# Autodesk Inventor assembly: Assembly1
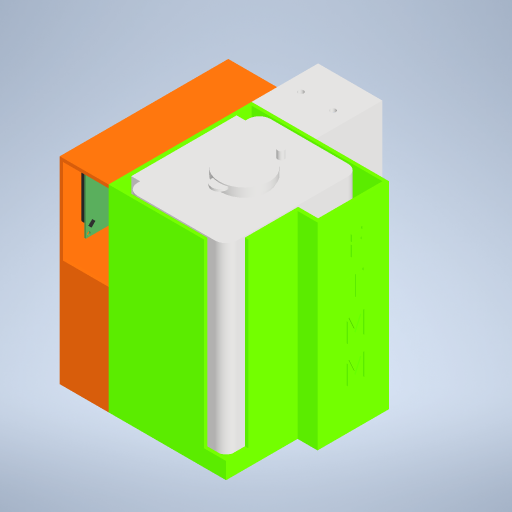
[picture p0: Inventor's stored thumbnail of the model, 512x512]
Saved by Autodesk Inventor 2023 (Build 270158000, 158)
## iProperties
Created: 2023-03-05
Part Number: Assembly1
Document SubType Name: Assembly
Designer: fatih
Author: fatih
## Documents named in this file (8)
- C:\Users\ACER\OneDrive - Universitas Airlangga\Kuliah\Pengmas-Hidroponik\Design\Assembly1.iam
- C:\Users\ACER\OneDrive - Universitas Airlangga\Kuliah\Pengmas-Hidroponik\Design\cover windshield.ipt
- C:\Users\ACER\OneDrive - Universitas Airlangga\Kuliah\Pengmas-Hidroponik\Design\windshield washer.ipt
- C:\Users\ACER\OneDrive - Universitas Airlangga\Kuliah\Pengmas-Hidroponik\Design\port side.ipt
- C:\Users\ACER\OneDrive - Universitas Airlangga\Kuliah\Pengmas-Hidroponik\Design\port plugin.ipt
- C:\Users\ACER\OneDrive - Universitas Airlangga\Kuliah\Pengmas-Hidroponik\Design\lcd-20x4-i2c-1.snapshot.4\Lcd i2c.ipt
- C:\Users\ACER\OneDrive - Universitas Airlangga\Kuliah\Pengmas-Hidroponik\Design\cover lcd.ipt
- C:\Users\ACER\OneDrive - Universitas Airlangga\Kuliah\Pengmas-Hidroponik\Design\back side.ipt
## Components (8 placed, 7 different names)
1. cover windshield:1 — Mate:1, Mate:2, Flush:1, Flush:2, Mate:6, Flush:3, Flush:4, Mate:10
2. windshield washer:1 — Mate:1, Mate:2
3. port side:1 — Flush:1, Flush:2, Mate:3, Mate:4, Mate:5, Mate:6, Mate:12
4. port plugin:1 — Mate:3, Mate:4, Mate:5
5. Lcd i2c:1 — Mate:7, Mate:8, Mate:9
6. cover lcd:1 — Mate:7, Mate:8, Mate:9, Flush:3, Flush:4, Mate:10, Mate:11, Flush:5
7. back side:1 — Mate:11, Flush:5, Mate:12, Flush:6
8. Lcd i2c:2 — Flush:6
## Relationships (18: Mate 12, Flush 6)
- Mate:1: cover windshield:1 ↔ windshield washer:1
- Mate:2: cover windshield:1 ↔ windshield washer:1
- Flush:1: cover windshield:1 ↔ port side:1
- Flush:2: cover windshield:1 ↔ port side:1
- Mate:3: port side:1 ↔ port plugin:1
- Mate:4: port side:1 ↔ port plugin:1
- Mate:5: port side:1 ↔ port plugin:1
- Mate:6: cover windshield:1 ↔ port side:1
- Mate:7: Lcd i2c:1 ↔ cover lcd:1
- Mate:8: Lcd i2c:1 ↔ cover lcd:1
- Mate:9: Lcd i2c:1 ↔ cover lcd:1
- Flush:3: cover windshield:1 ↔ cover lcd:1
- Flush:4: cover windshield:1 ↔ cover lcd:1
- Mate:10: cover windshield:1 ↔ cover lcd:1
- Mate:11: cover lcd:1 ↔ back side:1
- Flush:5: cover lcd:1 ↔ back side:1
- Mate:12: port side:1 ↔ back side:1
- Flush:6 (-3 mm): back side:1 ↔ Lcd i2c:2
